# Autodesk Inventor assembly: Daumen_Baugruppe
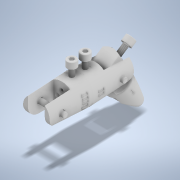
[picture p0: Inventor's stored thumbnail of the model, 180x180]
Saved by Autodesk Inventor 2021 (Build 250183000, 183)
## iProperties
Created: 2021-05-01
Part Number: Daumen_Baugruppe
Document SubType Name: Assembly
Designer: Maxim
Author: Maxim
## Documents named in this file (7)
- D:\MEDS Studium\4. Semester\Informatik IV\Bionic Hand Version 1.1\Daumen_Baugruppe.iam
- D:\MEDS Studium\4. Semester\Informatik IV\Bionic Hand Version 1.1\Fingerteil_1.ipt
- D:\MEDS Studium\4. Semester\Informatik IV\Bionic Hand Version 1.1\Fingerteil_2.ipt
- D:\MEDS Studium\4. Semester\Informatik IV\Bionic Hand Version 1.1\din_en_iso_4762_m3x10.ipt
- D:\MEDS Studium\4. Semester\Informatik IV\Bionic Hand Version 1.1\stift_iso_2338-3m6x20-a1.ipt
- D:\MEDS Studium\4. Semester\Informatik IV\Bionic Hand Version 1.1\din_en_iso_4762_m3x8.ipt
- D:\MEDS Studium\4. Semester\Informatik IV\Bionic Hand Version 1.1\Fingerteil_3_Daumen.ipt
## Components (8 placed, 6 different names)
1. Fingerteil_1:1 — Passend:5, Passend:6, Passend:12, Passend:17, Zylindrisch:1
2. Fingerteil_2:1 — Fluchtend:16, Passend:15, Passend:16, Passend:17, Zylindrisch:1, Passend:20, Passend:21, Passend:23
3. Fingerteil_3_Daumen:1 — Passend:13, Fluchtend:15, Passend:15, Passend:16, Passend:18, Passend:22, Passend:24
4. din_en_iso_4762_m3x10:1 — Passend:5, Passend:6
5. din_en_iso_4762_m3x8:1 — Passend:21, Passend:23
6. din_en_iso_4762_m3x8:2 — Passend:22, Passend:24
7. stift_iso_2338-3m6x20-a1:1 — Passend:12, Passend:20
8. stift_iso_2338-3m6x20-a1:2 — Passend:18, Passend:19
## Relationships (17: Mate 14, Flush 2, CylindricalJoint 1)
- Passend:5 [Mate]: Fingerteil_1:1 ↔ din_en_iso_4762_m3x10:1
- Passend:6 [Mate]: Fingerteil_1:1 ↔ din_en_iso_4762_m3x10:1
- Passend:12 [Mate] (-10 mm): Fingerteil_1:1 ↔ stift_iso_2338-3m6x20-a1:1
- Passend:13 [Mate]: Fingerteil_3_Daumen:1
- Fluchtend:15 [Flush]: Fingerteil_3_Daumen:1
- Fluchtend:16 [Flush]: Fingerteil_2:1
- Passend:15 [Mate]: Fingerteil_2:1 ↔ Fingerteil_3_Daumen:1
- Passend:16 [Mate]: Fingerteil_2:1 ↔ Fingerteil_3_Daumen:1
- Passend:17 [Mate] (0.2 mm): Fingerteil_1:1 ↔ Fingerteil_2:1
- Zylindrisch:1 [CylindricalJoint]: Fingerteil_1:1 ↔ Fingerteil_2:1
- Passend:18 [Mate]: Fingerteil_3_Daumen:1 ↔ stift_iso_2338-3m6x20-a1:2
- Passend:19 [Mate] (10 mm): stift_iso_2338-3m6x20-a1:2
- Passend:20 [Mate]: Fingerteil_2:1 ↔ stift_iso_2338-3m6x20-a1:1
- Passend:21 [Mate]: Fingerteil_2:1 ↔ din_en_iso_4762_m3x8:1
- Passend:22 [Mate]: Fingerteil_3_Daumen:1 ↔ din_en_iso_4762_m3x8:2
- Passend:23 [Mate]: Fingerteil_2:1 ↔ din_en_iso_4762_m3x8:1
- Passend:24 [Mate]: Fingerteil_3_Daumen:1 ↔ din_en_iso_4762_m3x8:2
